# Autodesk Inventor assembly: Laser w/ silver
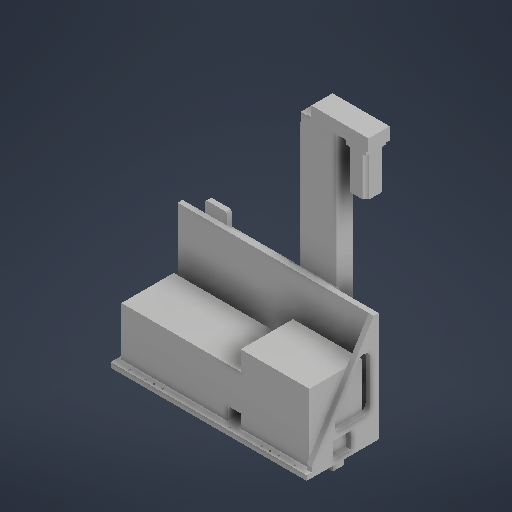
[picture p0: Inventor's stored thumbnail of the model, 512x512]
Saved by Autodesk Inventor 2025 (Build 290162000, 162)
## iProperties
Created: 2024-06-05
Part Number: Laser w/ silver
Document SubType Name: Assembly
Designer: AdminForWorker
Title: Laser w/ silver v4
Author: AdminForWorker
## Documents named in this file (3)
- C:\Users\mayhe\OneDrive\Documents\GitHub\In-situ-monitoring-of-powder-bed-fusion-additive-manufacturing\Laser Bed Fusion Printer CAD\Laser w_ silver v4.iam
- C:\Users\mayhe\OneDrive\Documents\GitHub\In-situ-monitoring-of-powder-bed-fusion-additive-manufacturing\Laser Bed Fusion Printer CAD\overhead laser unit v1.ipt
- C:\Users\mayhe\OneDrive\Documents\GitHub\In-situ-monitoring-of-powder-bed-fusion-additive-manufacturing\Laser Bed Fusion Printer CAD\Part4.ipt
## Components (2 placed, 2 different names)
1. overhead laser unit v1:1 — Mate:1
2. Part4 — Mate:1
## Relationships (1: Mate 1)
- Mate:1: overhead laser unit v1:1 ↔ Part4
